# Autodesk Inventor assembly: ASY Disk Micro filter v2.0
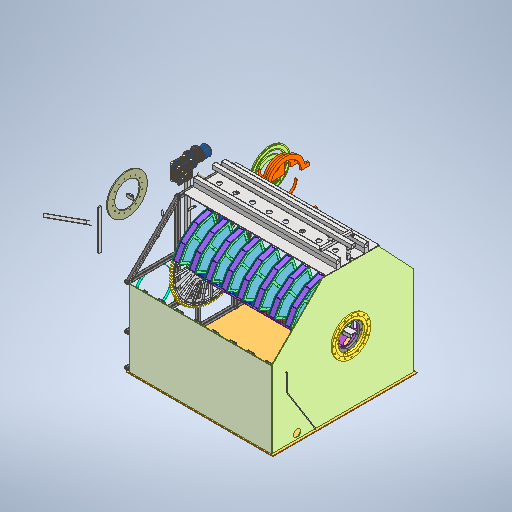
[picture p0: Inventor's stored thumbnail of the model, 512x512]
Saved by Autodesk Inventor 2026.2 (Build 302298000, 298)
## iProperties
Created: 2023-08-31
Part Number: ASY Disk Micro filter v2.0
Document SubType Name: Assembly
Designer: admin
Stock Number: Дисковый_Фильтр
Author: admin
## Documents named in this file (45)
- C:\Users\admin\Documents\Inventor\DMF-Disk-Micro-Filter\ASY 000 ДМФ Disk Micro filter v2.0.iam
- C:\Users\admin\Documents\Inventor\DMF-Disk-Micro-Filter\Left wall v2.0.ipt
- C:\Users\admin\Documents\Inventor\DMF-Disk-Micro-Filter\Wall right v2.0.ipt
- C:\Users\admin\Documents\Inventor\DMF-Disk-Micro-Filter\DF1.03 Wall bottom v2.0.ipt
- C:\Users\admin\Documents\Inventor\DMF-Disk-Micro-Filter\DF1.04 Wall face v2.0.ipt
- C:\Users\admin\Documents\Inventor\DMF-Disk-Micro-Filter\ДМФ 021 кольцо прижимное нос v2.0.ipt
- C:\Users\admin\Documents\Inventor\DMF-Disk-Micro-Filter\ДМФ 000 размеры v2.0.ipt
- C:\Users\admin\Documents\Inventor\DMF-Disk-Micro-Filter\ДМФ 032 крышка Нос v2.0.ipt
- C:\Users\admin\Documents\Inventor\DMF-Disk-Micro-Filter\ДМФ 091 Постель НОС v2.0.ipt
- C:\Users\admin\Documents\Inventor\DMF-Disk-Micro-Filter\ДМФ 022 кольцо прижимное корма v2.0.ipt
- C:\Users\admin\Documents\Inventor\DMF-Disk-Micro-Filter\ДМФ 093 Постель КОРМА v2.0.ipt
- C:\Users\admin\Documents\Inventor\DMF-Disk-Micro-Filter\ДМФ 092 Коромысло КОРМА v2.0.ipt
- C:\Users\admin\Documents\Inventor\DMF-Disk-Micro-Filter\ДМФ 055 труба илоотвода v2.0.ipt
- C:\Users\admin\Documents\Inventor\DMF-Disk-Micro-Filter\ДМФ 033 держатель лотка v2.0.ipt
- C:\Users\admin\Documents\Inventor\DMF-Disk-Micro-Filter\ASY ДМФ лоток 050 илоотвод v2.0.iam
- C:\Users\admin\Documents\Inventor\DMF-Disk-Micro-Filter\ДМФ 092 Коромысло НОС v2.0.ipt
- C:\Users\admin\Documents\Inventor\DMF-Disk-Micro-Filter\ДМФ 066 Гребенка v2.0.ipt
- C:\Users\admin\Documents\Inventor\DMF-Disk-Micro-Filter\ДМФ 025 кольцо прижимное корма наружное v2.0.ipt
- C:\Users\admin\Documents\Inventor\DMF-Disk-Micro-Filter\ДМФ 067 крышка v2.0.ipt
- C:\Users\admin\Documents\Inventor\DMF-Disk-Micro-Filter\ДМФ 081 труба форсунки v2.0.ipt
- C:\Users\admin\Documents\Inventor\DMF-Disk-Micro-Filter\ASY Обрешетка лицевая стенка.iam
- C:\Users\admin\Documents\Inventor\DMF-Disk-Micro-Filter\Вал ведущей шестерни.ipt
- C:\Users\admin\Documents\Inventor\DMF-Disk-Micro-Filter\Корпусный подшипник D35.ipt
- C:\Users\admin\Documents\Inventor\DMF-Disk-Micro-Filter\Мотор-редуктор NMRV 090(80B5).ipt
- C:\Users\admin\Documents\Inventor\DMF-Disk-Micro-Filter\DMF pancake.ipt
- C:\Users\admin\Documents\Inventor\DMF-Disk-Micro-Filter\Нога для постели.ipt
- C:\Users\admin\Documents\Inventor\DMF-Disk-Micro-Filter\Нога для постели №2.ipt
- C:\Users\admin\Documents\Inventor\DMF-Disk-Micro-Filter\ДМФ 092 Постель НОС v2.0.ipt
- C:\Users\admin\Documents\Inventor\DMF-Disk-Micro-Filter\ДМФ 094 Постель НОС крепление v2.0.ipt
- C:\Users\admin\Documents\Inventor\DMF-Disk-Micro-Filter\DMF Hat 2.0.ipt
- C:\Users\admin\Documents\Inventor\DMF-Disk-Micro-Filter\DMF Flange exit 2.0.ipt
- C:\Users\admin\Documents\Inventor\DMF-Disk-Micro-Filter\Барабан v2.1\ASY ДМФ 0100 Барабан v2.1.iam
- C:\Users\admin\Documents\Inventor\DMF-Disk-Micro-Filter\Барабан v2.1\DMF flange small gear.ipt
- C:\Users\admin\Documents\Inventor\DMF-Disk-Micro-Filter\Барабан v2.1\DMF small gear.ipt
- C:\Users\admin\Documents\Inventor\DMF-Disk-Micro-Filter\DMF Support ring tail.ipt
- C:\Users\admin\Documents\Inventor\DMF-Disk-Micro-Filter\DMF 082 коллектор болванка.ipt
- C:\Users\admin\Documents\Inventor\DMF-Disk-Micro-Filter\Барабан v2.1\DMF 2.1 Пластина паза маленькая.ipt
- C:\Users\admin\Documents\Inventor\DMF-Disk-Micro-Filter\Барабан v2.1\DMF 01 12 Барабан усилитель v2.1.ipt
- C:\Users\admin\Documents\Inventor\DMF-Disk-Micro-Filter\Барабан v2.1\DMF 2.1 01 45 Gear ring 5.ipt
- C:\Users\admin\Documents\Inventor\DMF-Disk-Micro-Filter\Барабан v2.1\DMF 2.1 01 46 Gear axis wheel 6.ipt
- C:\Users\admin\Documents\Inventor\DMF-Disk-Micro-Filter\Барабан v2.1\DMF 01 13 Барабан усилитель v2.1.ipt
- C:\Users\admin\Documents\Inventor\DMF-Disk-Micro-Filter\ДМФ 01 12 Барабан усилитель.ipt
- C:\Users\admin\Documents\Inventor\DMF-Disk-Micro-Filter\ДМФ 01 15 Барабан усилитель борта.ipt
- C:\Users\admin\Documents\Inventor\DMF-Disk-Micro-Filter\ДМФ 01 15 Барабан усилитель борта_CPY.ipt
- C:\Users\admin\Documents\Inventor\DMF-Disk-Micro-Filter\Барабан v2.1\DMF flange small gear 2.ipt
## Components (45 placed, 45 different names)
1. ДМФ 000 размеры v2.0.ipt:1
2. Left wall v2.0.ipt:1 — Flush:4, Mate:1, Flush:6, Flush:7, Flush:9, Mate:4, Flush:26, Flush:27, Mate:25, Rigid:16, Rigid:27, Rotational:19, Rotational:21
3. Wall right v2.0.ipt:1 — Flush:24, Rigid:16, Rigid:32, Mate:32
4. DF1.03 Wall bottom v2.0.ipt:1 — Mate:1, Flush:6, Flush:7, Mate:3, Flush:11, Mate:24, Mate:30
5. DF1.04 Wall face v2.0.ipt:1 — Flush:9, Mate:3, Mate:4, Flush:10, Angle:1
6. ДМФ 021 кольцо прижимное нос v2.0.ipt:1
7. ДМФ 032 крышка Нос v2.0.ipt:1
8. ДМФ 091 Постель НОС v2.0.ipt:1
9. ДМФ 022 кольцо прижимное корма v2.0.ipt:1
10. ДМФ 093 Постель КОРМА v2.0.ipt:1
11. ДМФ 092 Коромысло КОРМА v2.0.ipt:1
12. ДМФ 055 труба илоотвода v2.0.ipt:1 — Rigid:26, Cylindrical:30
13. ASY ДМФ лоток 050 илоотвод v2.0.iam:1 [sub-assembly]
14. ДМФ 092 Коромысло НОС v2.0.ipt:1
15. ДМФ 066 Гребенка v2.0.ipt:1 — Flush:22, Angle:1, Mate:24
16. ДМФ 025 кольцо прижимное корма наружное v2.0.ipt:1
17. ASY Обрешетка лицевая стенка.iam:1 [sub-assembly] — Flush:26, Flush:27, Mate:25
18. Вал ведущей шестерни.ipt:1 — Rotational:22, Rigid:36
19. Корпусный подшипник D35.ipt:1
20. Мотор-редуктор NMRV 090(80B5).ipt:1
21. DMF pancake.ipt:1 — Rigid:27, Rigid:28
22. Нога для постели.ipt:1
23. Нога для постели №2.ipt:1
24. ДМФ 092 Постель НОС v2.0.ipt:1
25. ДМФ 094 Постель НОС крепление v2.0.ipt:2
26. DMF Hat 2.0.ipt:1 — Rigid:28, Cylindrical:30
27. DMF Flange exit 2.0.ipt:1 — Rigid:26
28. DMF 01 12 Барабан усилитель v2.1.ipt:2
29. ДМФ 01 15 Барабан усилитель борта.ipt:4 — Mate:34, Mate:35
30. ДМФ 01 12 Барабан усилитель.ipt:2
31. DMF 2.1 01 46 Gear axis wheel 6.ipt:1
32. ДМФ 067 крышка v2.0.ipt:1 — Flush:24, Mate:32, Mate:33, Flush:35, Mate:36, Mate:37
33. DMF 2.1 01 45 Gear ring 5.ipt:1 — Rotational:21
34. DMF 01 13 Барабан усилитель v2.1.ipt:2
35. ASY ДМФ 0100 Барабан v2.1:1 [sub-assembly] — Rotational:17, Rotational:20
36. flange small gear:1 — Rigid:35, Rigid:36
37. DMF small gear:1 — Rotational:19, Rotational:22
38. DMF Support ring tail:1 — Rigid:32, Rotational:17, Rotational:20
39. DMF 082 коллектор болванка:1 — Rigid:33, Rigid:34, Mate:33, Mate:34, Mate:35, Flush:35
40. DMF 2.1 Пластина паза маленькая:1
41. ДМФ 081 труба форсунки v2.0:2 — Rigid:34
42. ДМФ 081 труба форсунки v2.0.ipt:1 — Rigid:33
43. ДМФ 033 держатель лотка v2.0.ipt:1 — Mate:36, Flush:36
44. ДМФ 01 15 Барабан усилитель борта_CPY:1 — Mate:37, Flush:36
45. DMF flange small gear 2:1 — Rigid:35
## Relationships (41: Mate 13, Flush 12, WeldJoint 9, RevoluteJoint 5, Angle 1, CylindricalJoint 1)
- Flush:4: Left wall v2.0.ipt:1
- Mate:1: Left wall v2.0.ipt:1 ↔ DF1.03 Wall bottom v2.0.ipt:1
- Flush:6 (15 mm): Left wall v2.0.ipt:1 ↔ DF1.03 Wall bottom v2.0.ipt:1
- Flush:7 (25 mm): Left wall v2.0.ipt:1 ↔ DF1.03 Wall bottom v2.0.ipt:1
- Flush:9: Left wall v2.0.ipt:1 ↔ DF1.04 Wall face v2.0.ipt:1
- Mate:3: DF1.03 Wall bottom v2.0.ipt:1 ↔ DF1.04 Wall face v2.0.ipt:1
- Mate:4: Left wall v2.0.ipt:1 ↔ DF1.04 Wall face v2.0.ipt:1
- Flush:10: DF1.04 Wall face v2.0.ipt:1
- Flush:11: DF1.03 Wall bottom v2.0.ipt:1
- [Mate]: ASY ДМФ лоток 050 илоотвод v2.0.iam:1
- Flush:22: ДМФ 066 Гребенка v2.0.ipt:1
- Angle:1 (180 deg): DF1.04 Wall face v2.0.ipt:1 ↔ ДМФ 066 Гребенка v2.0.ipt:1
- Mate:24: DF1.03 Wall bottom v2.0.ipt:1 ↔ ДМФ 066 Гребенка v2.0.ipt:1
- Flush:24: Wall right v2.0.ipt:1 ↔ ДМФ 067 крышка v2.0.ipt:1
- Flush:26: Left wall v2.0.ipt:1 ↔ ASY Обрешетка лицевая стенка.iam:1
- Flush:27: Left wall v2.0.ipt:1 ↔ ASY Обрешетка лицевая стенка.iam:1
- Mate:25: Left wall v2.0.ipt:1 ↔ ASY Обрешетка лицевая стенка.iam:1
- Rigid:16 [WeldJoint] (2140 mm): Left wall v2.0.ipt:1 ↔ Wall right v2.0.ipt:1
- Mate:30: DF1.03 Wall bottom v2.0.ipt:1
- Rigid:26 [WeldJoint]: ДМФ 055 труба илоотвода v2.0.ipt:1 ↔ DMF Flange exit 2.0.ipt:1
- Rigid:27 [WeldJoint]: Left wall v2.0.ipt:1 ↔ DMF pancake.ipt:1
- Rigid:28 [WeldJoint]: DMF pancake.ipt:1 ↔ DMF Hat 2.0.ipt:1
- Cylindrical:30: ДМФ 055 труба илоотвода v2.0.ipt:1 ↔ DMF Hat 2.0.ipt:1
- Rigid:32 [WeldJoint]: Wall right v2.0.ipt:1 ↔ DMF Support ring tail:1
- Rotational:17 [RevoluteJoint]: ASY ДМФ 0100 Барабан v2.1:1 ↔ DMF Support ring tail:1
- Rotational:19 [RevoluteJoint] (-32 mm): Left wall v2.0.ipt:1 ↔ DMF small gear:1
- Rotational:20 [RevoluteJoint]: ASY ДМФ 0100 Барабан v2.1:1 ↔ DMF Support ring tail:1
- Rigid:33 [WeldJoint]: DMF 082 коллектор болванка:1 ↔ ДМФ 081 труба форсунки v2.0.ipt:1
- Rigid:34 [WeldJoint]: DMF 082 коллектор болванка:1 ↔ ДМФ 081 труба форсунки v2.0:2
- Mate:32: Wall right v2.0.ipt:1 ↔ ДМФ 067 крышка v2.0.ipt:1
- Mate:33 (40 mm): ДМФ 067 крышка v2.0.ipt:1 ↔ DMF 082 коллектор болванка:1
- Rotational:21 [RevoluteJoint]: Left wall v2.0.ipt:1 ↔ DMF 2.1 01 45 Gear ring 5.ipt:1
- Mate:34: ДМФ 01 15 Барабан усилитель борта.ipt:4 ↔ DMF 082 коллектор болванка:1
- Mate:35: ДМФ 01 15 Барабан усилитель борта.ipt:4 ↔ DMF 082 коллектор болванка:1
- Flush:35: ДМФ 067 крышка v2.0.ipt:1 ↔ DMF 082 коллектор болванка:1
- Mate:36: ДМФ 067 крышка v2.0.ipt:1 ↔ ДМФ 033 держатель лотка v2.0.ipt:1
- Mate:37: ДМФ 067 крышка v2.0.ipt:1 ↔ ДМФ 01 15 Барабан усилитель борта_CPY:1
- Flush:36: ДМФ 033 держатель лотка v2.0.ipt:1 ↔ ДМФ 01 15 Барабан усилитель борта_CPY:1
- Rotational:22 [RevoluteJoint]: Вал ведущей шестерни.ipt:1 ↔ DMF small gear:1
- Rigid:35 [WeldJoint]: flange small gear:1 ↔ DMF flange small gear 2:1
- Rigid:36 [WeldJoint] (-25 mm): Вал ведущей шестерни.ipt:1 ↔ flange small gear:1
